# Autodesk Inventor assembly: Sandbox
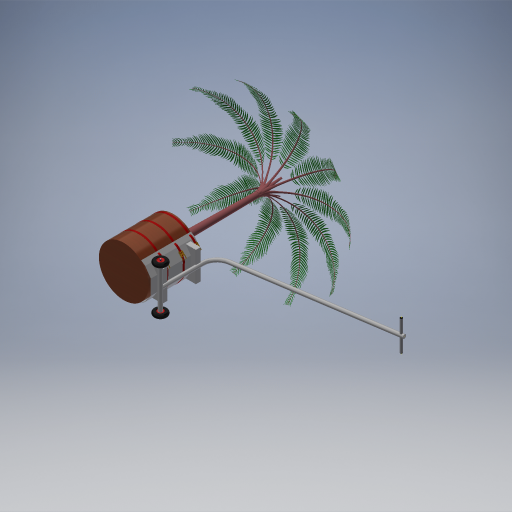
[picture p0: Inventor's stored thumbnail of the model, 512x512]
Saved by Autodesk Inventor 2023.2 (Build 272271000, 271)
## iProperties
Created: 2023-02-01
Part Number: Sandbox
Material: Generisch
Document SubType Name: Assembly
Designer: Raoul Messerli
Mass: 818109 g
Surface Area: 182177 cm^2
Volume: 770414 cm^3
Density: 1.06191 g/cm^3
Author: Raoul Messerli
## Documents named in this file (14)
- E:\GitHub\Pflanzenwagen\40_Realisieren\20_Inventor\40_Baugruppen\Sandbox.iam
- E:\GitHub\Pflanzenwagen\40_Realisieren\20_Inventor\10_Vorlage\Palme.iam
- E:\GitHub\Pflanzenwagen\40_Realisieren\20_Inventor\20_Einkaufteile\RatchetStrap\RatchetStrap\RatchetStrap.iam
- E:\GitHub\Pflanzenwagen\40_Realisieren\20_Inventor\30_Fertigungsteile\Blech1.ipt
- E:\GitHub\Pflanzenwagen\40_Realisieren\20_Inventor\20_Einkaufteile\RatchetStrap\Strap for Pflanzenwagen.ipt
- E:\GitHub\Pflanzenwagen\40_Realisieren\20_Inventor\20_Einkaufteile\Wheel.ipt
- E:\GitHub\Pflanzenwagen\40_Realisieren\20_Inventor\30_Fertigungsteile\Achse.ipt
- E:\GitHub\Pflanzenwagen\40_Realisieren\20_Inventor\30_Fertigungsteile\Rad Aufnahme.ipt
- E:\GitHub\Pflanzenwagen\40_Realisieren\20_Inventor\20_Einkaufteile\BN 161 1118811 prevailing torque type hex lock nut M20_Steel 6.ipt
- E:\GitHub\Pflanzenwagen\40_Realisieren\20_Inventor\30_Fertigungsteile\Hebel.ipt
- E:\GitHub\Pflanzenwagen\40_Realisieren\20_Inventor\30_Fertigungsteile\Halteblech.ipt
- E:\GitHub\Pflanzenwagen\40_Realisieren\20_Inventor\30_Fertigungsteile\Deckel.ipt
- E:\GitHub\Pflanzenwagen\40_Realisieren\20_Inventor\30_Fertigungsteile\Griff.ipt
- E:\GitHub\Pflanzenwagen\40_Realisieren\20_Inventor\20_Einkaufteile\Round_sliders.ipt
## Components (22 placed, 13 different names)
1. Strap for Pflanzenwagen:1 — Passend:7, Fluchtend:9, Passend:8
2. Strap for Pflanzenwagen:2 — Passend:9, Fluchtend:10, Passend:10
3. Strap for Pflanzenwagen:3 — Passend:11, Fluchtend:11, Passend:12
4. Palme:1 [sub-assembly] — Fluchtend:1, Fluchtend:2, Tangential:1, Fluchtend:3, Fluchtend:4, Fluchtend:5, Passend:13, Passend:14, Fluchtend:12, Passend:30, Winkel:1
5. Blech1:1 — Fluchtend:1, Fluchtend:2, Tangential:1, Fluchtend:6, Passend:1, Passend:2, Passend:3, Fluchtend:7, Passend:4, Passend:5, Fluchtend:8, Passend:6, Passend:10, Winkel:2, Fluchtend:15
6. RatchetStrap:1 [sub-assembly] — Fluchtend:6, Passend:1, Passend:2, Passend:8
7. RatchetStrap:2 [sub-assembly] — Passend:3, Fluchtend:7, Passend:4
8. RatchetStrap:3 [sub-assembly] — Passend:5, Fluchtend:8, Passend:6, Passend:12
9. Achse:1 — Passend:13, Passend:14, Fluchtend:12, Passend:31, Tangential:2
10. Rad Aufnahme:1 — Passend:21, Passend:24, Passend:29
11. Rad Aufnahme:2 — Passend:22, Passend:23
12. Wheel:1 — Passend:21, Passend:24
13. Wheel:2 — Passend:22, Passend:23, Passend:28
14. BN 161 1118811 prevailing torque type hex lock nut M20_Steel 6:2 — Passend:28
15. BN 161 1118811 prevailing torque type hex lock nut M20_Steel 6:3 — Passend:29
16. Hebel:1 — Passend:30, Passend:31, Winkel:1, Fluchtend:13, Fluchtend:14, Passend:32, Passend:33, Passend:34, Passend:35, Passend:36
17. Halteblech:1 — Fluchtend:13, Fluchtend:14, Tangential:2
18. Halteblech:2 — Passend:32, Winkel:2, Fluchtend:15
19. Deckel:1 — Passend:33, Passend:34
20. Griff:1 — Passend:35, Passend:36, Passend:38, Passend:39, Passend:40, Passend:41
21. Round_sliders:1 — Passend:39, Passend:40
22. Round_sliders:2 — Passend:38, Passend:41
## Relationships (50: Mate 31, Flush 15, Tangent 2, Angle 2)
- Fluchtend:1 [Flush]: Palme:1 ↔ Blech1:1
- Fluchtend:2 [Flush]: Palme:1 ↔ Blech1:1
- Tangential:1: Palme:1 ↔ Blech1:1
- Fluchtend:3 [Flush]: Palme:1
- Fluchtend:4 [Flush]: Palme:1
- Fluchtend:5 [Flush]: Palme:1
- Fluchtend:6 [Flush]: Blech1:1 ↔ RatchetStrap:1
- Passend:1 [Mate]: Blech1:1 ↔ RatchetStrap:1
- Passend:2 [Mate]: Blech1:1 ↔ RatchetStrap:1
- Passend:3 [Mate]: Blech1:1 ↔ RatchetStrap:2
- Fluchtend:7 [Flush]: Blech1:1 ↔ RatchetStrap:2
- Passend:4 [Mate]: Blech1:1 ↔ RatchetStrap:2
- Passend:5 [Mate]: Blech1:1 ↔ RatchetStrap:3
- Fluchtend:8 [Flush]: Blech1:1 ↔ RatchetStrap:3
- Passend:6 [Mate]: Blech1:1 ↔ RatchetStrap:3
- Passend:7 [Mate]: Strap for Pflanzenwagen:1
- Fluchtend:9 [Flush]: Strap for Pflanzenwagen:1
- Passend:8 [Mate]: Strap for Pflanzenwagen:1 ↔ RatchetStrap:1
- Passend:9 [Mate]: Strap for Pflanzenwagen:2
- Fluchtend:10 [Flush]: Strap for Pflanzenwagen:2
- Passend:10 [Mate]: Strap for Pflanzenwagen:2 ↔ Blech1:1
- Passend:11 [Mate]: Strap for Pflanzenwagen:3
- Fluchtend:11 [Flush]: Strap for Pflanzenwagen:3
- Passend:12 [Mate]: Strap for Pflanzenwagen:3 ↔ RatchetStrap:3
- Passend:13 [Mate] (-420 mm): Palme:1 ↔ Achse:1
- Passend:14 [Mate] (400 mm): Palme:1 ↔ Achse:1
- Passend:21 [Mate]: Rad Aufnahme:1 ↔ Wheel:1
- Passend:22 [Mate]: Rad Aufnahme:2 ↔ Wheel:2
- Passend:23 [Mate]: Rad Aufnahme:2 ↔ Wheel:2
- Passend:24 [Mate]: Rad Aufnahme:1 ↔ Wheel:1
- Passend:28 [Mate]: Wheel:2 ↔ BN 161 1118811 prevailing torque type hex lock nut M20_Steel 6:2
- Passend:29 [Mate]: Rad Aufnahme:1 ↔ BN 161 1118811 prevailing torque type hex lock nut M20_Steel 6:3
- Fluchtend:12 [Flush] (-650 mm): Palme:1 ↔ Achse:1
- Passend:30 [Mate]: Palme:1 ↔ Hebel:1
- Passend:31 [Mate]: Achse:1 ↔ Hebel:1
- Winkel:1 [Angle] (0 deg): Palme:1 ↔ Hebel:1
- Fluchtend:13 [Flush]: Hebel:1 ↔ Halteblech:1
- Fluchtend:14 [Flush]: Hebel:1 ↔ Halteblech:1
- Tangential:2: Achse:1 ↔ Halteblech:1
- Passend:32 [Mate]: Hebel:1 ↔ Halteblech:2
- Winkel:2 [Angle] (0 deg): Blech1:1 ↔ Halteblech:2
- Fluchtend:15 [Flush] (100 mm): Blech1:1 ↔ Halteblech:2
- Passend:33 [Mate]: Hebel:1 ↔ Deckel:1
- Passend:34 [Mate]: Hebel:1 ↔ Deckel:1
- Passend:35 [Mate]: Hebel:1 ↔ Griff:1
- Passend:36 [Mate]: Hebel:1 ↔ Griff:1
- Passend:38 [Mate]: Griff:1 ↔ Round_sliders:2
- Passend:39 [Mate]: Griff:1 ↔ Round_sliders:1
- Passend:40 [Mate]: Griff:1 ↔ Round_sliders:1
- Passend:41 [Mate]: Griff:1 ↔ Round_sliders:2
